# Autodesk Inventor assembly: Estrutura do Trem
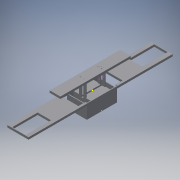
[picture p0: Inventor's stored thumbnail of the model, 180x180]
Saved by Autodesk Inventor 2018 (Build 220112000, 112)
## iProperties
Created: 2018-02-27
Part Number: Estrutura do Trem
Document SubType Name: Assembly
Designer: matheus
Author: matheus
## Documents named in this file (4)
- Z:\Estrutura do Trem.iam
- Z:\Base_trem.ipt
- Z:\Placa do Circuito.ipt
- Z:\Suporte_motor.ipt
## Components (3 placed, 3 different names)
1. Base_trem:1 — Mate:1
2. Suporte_motor:1 — Mate:1, Mate:2
3. Placa do Circuito:1 — Mate:2
## Relationships (2: Mate 2)
- Mate:1: Base_trem:1 ↔ Suporte_motor:1
- Mate:2: Suporte_motor:1 ↔ Placa do Circuito:1
